# Autodesk Inventor assembly: MTG eixorodaencode
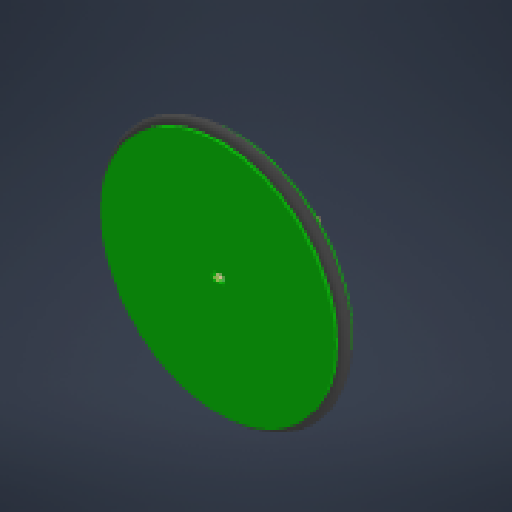
[picture p0: Inventor's stored thumbnail of the model, 512x512]
Saved by Autodesk Inventor 2026 (Build 300175000, 175)
## iProperties
Created: 2025-09-18
Part Number: MTG eixorodaencode
Document SubType Name: Assembly
Designer: Administrador
Author: Administrador
## Documents named in this file (5)
- C:\Users\pregu\OneDrive\Documentos\Carro 8.5\MTG eixorodaencode.iam
- C:\Users\pregu\OneDrive\Documentos\Carro 8.5\Motor Amarelo\Parte 2.ipt
- C:\Users\pregu\OneDrive\Documentos\Carro 8.5\Encoder-HC-020K\Encoder Disco-Novo-12-furos-04.ipt
- C:\Users\pregu\OneDrive\Documentos\Carro 8.5\Rodinha-02.ipt
- C:\Users\pregu\OneDrive\Documentos\Carro 8.5\Rodinha-Borracha.ipt
## Components (4 placed, 4 different names)
1. Parte 2:1 — Coincidente:3, Coincidente:4, Coincidente:5, Alinhado:2, Coincidente:8, Coincidente:14, Alinhado:3
2. Encoder Disco-Novo-12-furos-04:1 — Coincidente:14, Alinhado:3
3. Rodinha-02:1 — Coincidente:1, Coincidente:2, Coincidente:3, Coincidente:4, Coincidente:5, Coincidente:8
4. Rodinha-Borracha:1 — Coincidente:1, Coincidente:2
## Relationships (9: Mate 7, Flush 2)
- Coincidente:1 [Mate]: Rodinha-02:1 ↔ Rodinha-Borracha:1
- Coincidente:2 [Mate] (4.5 mm): Rodinha-02:1 ↔ Rodinha-Borracha:1
- Coincidente:3 [Mate]: Parte 2:1 ↔ Rodinha-02:1
- Coincidente:4 [Mate]: Parte 2:1 ↔ Rodinha-02:1
- Coincidente:5 [Mate]: Parte 2:1 ↔ Rodinha-02:1
- Alinhado:2 [Flush]: Parte 2:1
- Coincidente:8 [Mate]: Parte 2:1 ↔ Rodinha-02:1
- Coincidente:14 [Mate]: Parte 2:1 ↔ Encoder Disco-Novo-12-furos-04:1
- Alinhado:3 [Flush]: Parte 2:1 ↔ Encoder Disco-Novo-12-furos-04:1
